# Autodesk Inventor assembly: ArmAndMotorV02
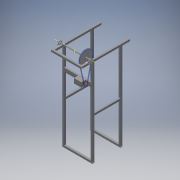
[picture p0: Inventor's stored thumbnail of the model, 180x180]
Saved by Autodesk Inventor 2018.2 (Build 222227000, 227)
## iProperties
Created: 2018-02-08
Part Number: ArmAndMotorV02
Document SubType Name: Assembly
Designer: steele
Author: steele
## Documents named in this file (15)
- D:\snobotics\CAD-Development\robSteele\2018-FRC\Arm\ArmAndMotorV02.iam
- D:\snobotics\CAD-Development\robSteele\2018-FRC\Arm\1x16_25-rectangular.ipt
- D:\snobotics\CAD-Development\robSteele\2018-FRC\Arm\1x2x14_25-rectangular.ipt
- D:\snobotics\CAD-Development\robSteele\2018-FRC\Arm\AM Rev 3209 Motor Mount.ipt
- D:\snobotics\CAD-Development\robSteele\2018-FRC\Arm\BaneBot220GearBox.ipt
- D:\snobotics\CAD-Development\robSteele\2018-FRC\Arm\hexExtrusion.ipt
- D:\snobotics\CAD-Development\robSteele\2018-FRC\Arm\ArmAndMotorV02\Design Accelerator\Chain Drive1.iam
- D:\snobotics\CAD-Development\robSteele\2018-FRC\backOfRobot.ipt
- D:\snobotics\CAD-Development\robSteele\2018-FRC\Arm\1x14-rectangular.ipt
- D:\snobotics\CAD-Development\robSteele\2018-FRC\Arm\1x25-topPost.ipt
- D:\snobotics\CAD-Development\robSteele\2018-FRC\Arm\1x46-rectangular.ipt
- D:\snobotics\CAD-Development\robSteele\2018-FRC\Arm\ArmAndMotorV02\Design Accelerator\Bolted Connection5.iam
- D:\snobotics\CAD-Development\robSteele\2018-FRC\Arm\ArmAndMotorV02\Design Accelerator\Bolted Connection6.iam
- D:\snobotics\CAD-Development\robSteele\2018-FRC\Arm\ArmAndMotorV02\Design Accelerator\Bolted Connection7.iam
- D:\snobotics\CAD-Development\robSteele\2018-FRC\Arm\ArmAndMotorV02\Design Accelerator\Bolted Connection8.iam
## Components (22 placed, 11 different names)
1. 1x46-rectangular:1 — Flush:1, Flush:2, Mate:1, Mate:4, Flush:6, Flush:8, Mate:7, Flush:18, Mate:31, Flush:22
2. 1x46-rectangular:2 — Flush:1, Flush:2, Mate:1, Flush:3, Flush:4, Mate:2, Mate:3, Flush:5, Flush:7, Mate:5, Flush:9, Mate:9
3. 1x16_25-rectangular:1 — Flush:3, Flush:4, Mate:2, Flush:21
4. 1x25-topPost:1 — Mate:4, Flush:6, Flush:8, Mate:6, Flush:11, Mate:13, Mate:14, Flush:16, Flush:20, Mate:32
5. 1x25-topPost:2 — Mate:3, Flush:5, Flush:7, Flush:10, Mate:8, Flush:12, Mate:11, Mate:12, Flush:15, Mate:18, Mate:34, Mate:35, Flush:24, Flush:25
6. 1x2x14_25-rectangular:1 — Mate:5, Flush:9, Flush:10, Flush:17, Mate:17
7. 1x46-rectangular:3 — Mate:6, Flush:11, Mate:7
8. 1x46-rectangular:4 — Mate:8, Flush:12, Mate:9, Mate:10, Flush:13, Flush:14, Mate:33, Flush:23
9. 1x16_25-rectangular:2 — Mate:10, Flush:13, Flush:14
10. AM Rev 3209 Motor Mount:1 — Mate:11, Mate:12, Flush:15, Mate:16, Flush:19, Mate:23, Mate:24
11. AM Rev 3209 Motor Mount:2 — Mate:13, Mate:14, Flush:16, Mate:25, Mate:26, Mate:27, Mate:28, Mate:29, Mate:30
12. BaneBot220GearBox:1 — Flush:17, Flush:18, Mate:17
13. hexExtrusion:1 — Mate:16, Flush:19
14. Chain Drive:1 [sub-assembly]
15. backOfRobot:1 — Mate:18, Flush:20, Flush:21
16. 1x14-rectangular:1 — Mate:33, Flush:23, Mate:34
17. 1x14-rectangular:2 — Mate:31, Flush:22, Mate:32
18. Bolted Connection:1 [sub-assembly] — Mate:25, Mate:26
19. Bolted Connection:3 [sub-assembly] — Mate:23, Mate:24
20. Bolted Connection:4 [sub-assembly] — Mate:27, Mate:28
21. Bolted Connection:5 [sub-assembly] — Mate:29, Mate:30
22. 1x16_25-rectangular:3 — Mate:35, Flush:24, Flush:25
## Relationships (55: Mate 30, Flush 25)
- Flush:1: 1x46-rectangular:1 ↔ 1x46-rectangular:2
- Flush:2: 1x46-rectangular:1 ↔ 1x46-rectangular:2
- Mate:1 (361.95 mm): 1x46-rectangular:1 ↔ 1x46-rectangular:2
- Flush:3: 1x46-rectangular:2 ↔ 1x16_25-rectangular:1
- Flush:4: 1x46-rectangular:2 ↔ 1x16_25-rectangular:1
- Mate:2: 1x46-rectangular:2 ↔ 1x16_25-rectangular:1
- Mate:3: 1x46-rectangular:2 ↔ 1x25-topPost:2
- Flush:5: 1x46-rectangular:2 ↔ 1x25-topPost:2
- Mate:4: 1x46-rectangular:1 ↔ 1x25-topPost:1
- Flush:6: 1x46-rectangular:1 ↔ 1x25-topPost:1
- Flush:7 (127 mm): 1x46-rectangular:2 ↔ 1x25-topPost:2
- Flush:8 (127 mm): 1x46-rectangular:1 ↔ 1x25-topPost:1
- Mate:5: 1x46-rectangular:2 ↔ 1x2x14_25-rectangular:1
- Flush:9: 1x46-rectangular:2 ↔ 1x2x14_25-rectangular:1
- Flush:10 (274.7518 mm): 1x25-topPost:2 ↔ 1x2x14_25-rectangular:1
- Mate:6: 1x25-topPost:1 ↔ 1x46-rectangular:3
- Flush:11: 1x25-topPost:1 ↔ 1x46-rectangular:3
- Mate:7 (355.6 mm): 1x46-rectangular:1 ↔ 1x46-rectangular:3
- Mate:8: 1x25-topPost:2 ↔ 1x46-rectangular:4
- Flush:12: 1x25-topPost:2 ↔ 1x46-rectangular:4
- Mate:9 (355.6 mm): 1x46-rectangular:2 ↔ 1x46-rectangular:4
- Mate:10: 1x46-rectangular:4 ↔ 1x16_25-rectangular:2
- Flush:13: 1x46-rectangular:4 ↔ 1x16_25-rectangular:2
- Flush:14: 1x46-rectangular:4 ↔ 1x16_25-rectangular:2
- Mate:11: 1x25-topPost:2 ↔ AM Rev 3209 Motor Mount:1
- Mate:12: 1x25-topPost:2 ↔ AM Rev 3209 Motor Mount:1
- Flush:15 (-50.8 mm): 1x25-topPost:2 ↔ AM Rev 3209 Motor Mount:1
- Mate:13: 1x25-topPost:1 ↔ AM Rev 3209 Motor Mount:2
- Mate:14: 1x25-topPost:1 ↔ AM Rev 3209 Motor Mount:2
- Flush:16 (-50.8 mm): 1x25-topPost:1 ↔ AM Rev 3209 Motor Mount:2
- Flush:17 (6.35 mm): 1x2x14_25-rectangular:1 ↔ BaneBot220GearBox:1
- Flush:18 (88.9 mm): 1x46-rectangular:1 ↔ BaneBot220GearBox:1
- Mate:16: AM Rev 3209 Motor Mount:1 ↔ hexExtrusion:1
- Flush:19 (25.4 mm): AM Rev 3209 Motor Mount:1 ↔ hexExtrusion:1
- Mate:17: 1x2x14_25-rectangular:1 ↔ BaneBot220GearBox:1
- Mate:18: 1x25-topPost:2 ↔ backOfRobot:1
- Flush:20 (92.075 mm): 1x25-topPost:1 ↔ backOfRobot:1
- Flush:21 (53.975 mm): 1x16_25-rectangular:1 ↔ backOfRobot:1
- Mate:23: AM Rev 3209 Motor Mount:1 ↔ Bolted Connection:3
- Mate:24: AM Rev 3209 Motor Mount:1 ↔ Bolted Connection:3
- Mate:25: AM Rev 3209 Motor Mount:2 ↔ Bolted Connection:1
- Mate:26: AM Rev 3209 Motor Mount:2 ↔ Bolted Connection:1
- Mate:27: AM Rev 3209 Motor Mount:2 ↔ Bolted Connection:4
- Mate:28: AM Rev 3209 Motor Mount:2 ↔ Bolted Connection:4
- Mate:29: AM Rev 3209 Motor Mount:2 ↔ Bolted Connection:5
- Mate:30: AM Rev 3209 Motor Mount:2 ↔ Bolted Connection:5
- Mate:31: 1x46-rectangular:1 ↔ 1x14-rectangular:2
- Flush:22: 1x46-rectangular:1 ↔ 1x14-rectangular:2
- Mate:32 (609.6 mm): 1x25-topPost:1 ↔ 1x14-rectangular:2
- Mate:33: 1x46-rectangular:4 ↔ 1x14-rectangular:1
- Flush:23: 1x46-rectangular:4 ↔ 1x14-rectangular:1
- Mate:34 (609.6 mm): 1x25-topPost:2 ↔ 1x14-rectangular:1
- Mate:35: 1x25-topPost:2 ↔ 1x16_25-rectangular:3
- Flush:24: 1x25-topPost:2 ↔ 1x16_25-rectangular:3
- Flush:25: 1x25-topPost:2 ↔ 1x16_25-rectangular:3
## Named parameters: backOfRobotToBearningBlock = 50.8 mm, fromTopOfFrameToTopOfMotorSupport = 274.7518 mm
